# Autodesk Inventor assembly: California_Corner_MIR_MIR
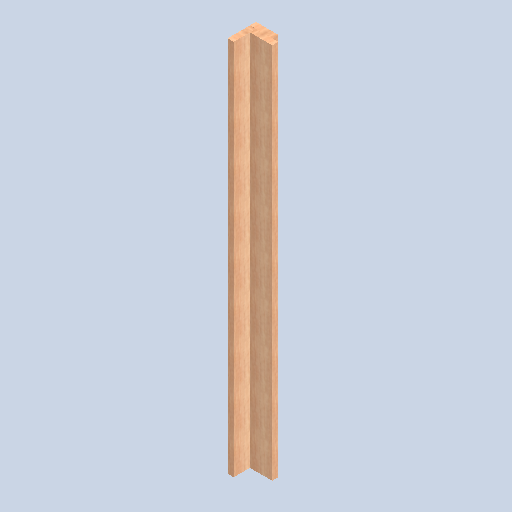
[picture p0: Inventor's stored thumbnail of the model, 512x512]
Saved by Autodesk Inventor 2025 (Build 290162010, 162A)
## iProperties
Created: 2024-09-15
Part Number: California_Corner_MIR_MIR
Document SubType Name: Assembly
Designer: Tom
Author: Tom
## Documents named in this file (2)
- C:\Users\Tom\Documents\Inventor\Mobility\Additional_Building\California_Corner_MIR_MIR.iam
- C:\Users\Tom\Documents\Inventor\Mobility\Additional_Building\Stud_With_Height_93_Inches_MIR_MIR.ipt
## Components (3 placed, 1 different names)
1. Stud_With_Height_93_Inches_MIR_MIR:1 — Mate:1, Flush:1, Flush:2, Mate:3, Flush:3
2. Stud_With_Height_93_Inches_MIR_MIR:2 — Mate:1, Flush:1, Flush:2, Mate:2
3. Stud_With_Height_93_Inches_MIR_MIR:3 — Mate:2, Mate:3, Flush:3
## Relationships (6: Mate 3, Flush 3)
- Mate:1: Stud_With_Height_93_Inches_MIR_MIR:1 ↔ Stud_With_Height_93_Inches_MIR_MIR:2
- Flush:1: Stud_With_Height_93_Inches_MIR_MIR:1 ↔ Stud_With_Height_93_Inches_MIR_MIR:2
- Flush:2: Stud_With_Height_93_Inches_MIR_MIR:1 ↔ Stud_With_Height_93_Inches_MIR_MIR:2
- Mate:2: Stud_With_Height_93_Inches_MIR_MIR:2 ↔ Stud_With_Height_93_Inches_MIR_MIR:3
- Mate:3: Stud_With_Height_93_Inches_MIR_MIR:1 ↔ Stud_With_Height_93_Inches_MIR_MIR:3
- Flush:3: Stud_With_Height_93_Inches_MIR_MIR:1 ↔ Stud_With_Height_93_Inches_MIR_MIR:3
